# Autodesk Inventor assembly: SE. Chasis DC
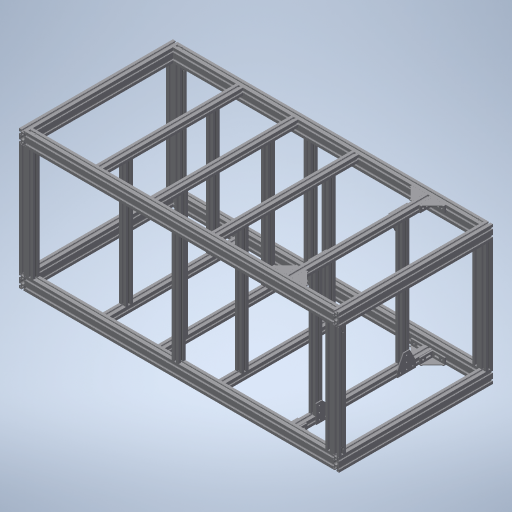
[picture p0: Inventor's stored thumbnail of the model, 512x512]
Saved by Autodesk Inventor 2024.2 (Build 282272000, 272)
## iProperties
Created: 2024-06-24
Part Number: SE. Chasis DC
Material: Genérico
Document SubType Name: Assembly
Designer: jd.castellanosq
Author: jd.castellanosq
## Documents named in this file (12)
- I:\MICROMECANICA\ALTAS ENERGIAS\Deteccion de Muones\Detectores centelladores\Partes Detector Centellador\SE Chasis DC\SE. Chasis DC.iam
- I:\MICROMECANICA\ALTAS ENERGIAS\Deteccion de Muones\Detectores centelladores\Partes Detectores centelladores\Chasis DC\Partes Chasis DC\Perfil 45X90.ipt
- I:\MICROMECANICA\ALTAS ENERGIAS\Deteccion de Muones\Detectores centelladores\Partes Detector Centellador\SE Chasis DC\Partes Chasis DC\Perfil 45X45\Perfil 45X45x910.ipt
- I:\MICROMECANICA\ALTAS ENERGIAS\Deteccion de Muones\Detectores centelladores\Partes Detectores centelladores\Chasis DC\Partes Chasis DC\Perfil 45X45.ipt
- I:\MICROMECANICA\ALTAS ENERGIAS\Deteccion de Muones\Detectores centelladores\Partes Detector Centellador\SE Chasis DC\Partes Chasis DC\Perfil 45X45\Perfil 45X45X720.ipt
- I:\MICROMECANICA\ALTAS ENERGIAS\Deteccion de Muones\Detectores centelladores\Partes Detector Centellador\SE Chasis DC\Partes Chasis DC\Accesorios perfileria\escuadra grande.ipt
- I:\MICROMECANICA\ALTAS ENERGIAS\Deteccion de Muones\Detectores centelladores\Partes Detector Centellador\SE Chasis DC\Partes Chasis DC\Accesorios perfileria\escuadra plana.ipt
- I:\MICROMECANICA\ALTAS ENERGIAS\Deteccion de Muones\Detectores centelladores\Partes Detector Centellador\SE Chasis DC\Partes Chasis DC\Accesorios perfileria\T.ipt
- I:\MICROMECANICA\ALTAS ENERGIAS\Deteccion de Muones\Detectores centelladores\Partes Detector Centellador\SE Chasis DC\Partes Chasis DC\Perfil 45X45\Perfil 45X45X810.ipt
- I:\MICROMECANICA\ALTAS ENERGIAS\Deteccion de Muones\Detectores centelladores\Partes Detector Centellador\SE Chasis DC\Partes Chasis DC\Perfil 45X90\Perfil 45X90x1000.ipt
- I:\MICROMECANICA\ALTAS ENERGIAS\Deteccion de Muones\Detectores centelladores\Partes Detector Centellador\SE Chasis DC\Partes Chasis DC\Perfil 45X90\Perfil 45X90x720.ipt
- I:\MICROMECANICA\ALTAS ENERGIAS\Deteccion de Muones\Detectores centelladores\Partes Detector Centellador\SE Chasis DC\Partes Chasis DC\Perfil 45X90\Perfil 45X90x1990.ipt
## Components (42 placed, 9 different names)
1. Perfil 45X90x1990:13 — Mate:65, Flush:83, Flush:84, Flush:85, Flush:86, Mate:66, Flush:92, Mate:71, Flush:94, Mate:72, Flush:108, Mate:82, Mate:91, Mate:99, Mate:114, Flush:131, Flush:138
2. Perfil 45X90x1000:17 — Mate:65, Flush:83, Flush:84, Flush:95, Flush:99, Mate:74
3. Perfil 45X90x1000:18 — Flush:85, Flush:86, Mate:66, Mate:67, Flush:87, Flush:88, Flush:93, Flush:97
4. Perfil 45X90x1990:21 — Mate:67, Flush:87, Flush:88, Flush:96, Mate:73, Flush:98, Flush:109, Flush:110, Mate:85, Mate:95, Mate:97, Mate:113, Flush:130, Mate:117
5. Perfil 45X45x910:39 — Flush:109
6. Perfil 45X45x910:40 — Flush:110, Mate:82
7. Perfil 45X45x910:41 — Flush:108, Flush:116, Mate:92, Mate:93, Mate:94, Flush:117, Mate:96, Flush:118, Mate:98, Flush:123, Flush:125
8. Perfil 45X45X810:45 — Flush:139
9. Perfil 45X45X810:46 — Flush:140
10. Perfil 45X45X810:47 — Mate:86, Mate:109, Mate:110, Mate:111
11. Perfil 45X45X810:48 — Mate:85, Mate:86, Mate:108, Flush:124, Mate:112, Flush:129
12. Perfil 45X45X810:49
13. Perfil 45X45X810:50
14. Perfil 45X90x1990:14 — Flush:106, Flush:107, Mate:78, Mate:101, Mate:102
15. Perfil 45X90x1000:19 — Flush:100, Flush:101, Mate:75, Mate:76, Flush:107, Mate:78
16. Perfil 45X90x1000:20 — Flush:103, Flush:104, Flush:105
17. Perfil 45X90x1990:28 — Mate:76, Flush:102, Mate:77, Flush:105, Flush:112, Mate:89, Mate:90, Mate:105, Mate:107, Mate:116
18. Perfil 45X90x720:9 — Flush:96, Flush:97, Mate:73, Flush:103, Flush:104
19. Perfil 45X90x720:10 — Flush:92, Mate:71, Flush:93
20. Perfil 45X90x720:11 — Flush:94, Mate:72, Flush:95, Flush:106
21. Perfil 45X90x720:12 — Flush:98, Flush:99, Mate:74, Flush:100, Flush:101, Mate:75, Flush:102, Mate:77
22. Perfil 45X45x910:42 — Mate:89
23. Perfil 45X45x910:43 — Flush:112, Flush:137
24. Perfil 45X45x910:44 — Mate:90, Flush:119, Mate:100, Flush:120, Mate:103, Flush:121, Mate:104, Flush:122, Mate:106, Flush:126, Flush:128
25. escuadra grande:1 — Flush:117, Mate:96, Mate:97
26. escuadra grande:2 — Mate:93, Mate:94, Mate:95
27. escuadra grande:3 — Flush:122, Mate:106, Mate:107
28. escuadra grande:4 — Flush:118, Mate:98, Mate:99
29. escuadra grande:5 — Flush:119, Mate:100, Mate:101
30. escuadra grande:6 — Flush:120, Mate:102, Mate:103
31. escuadra grande:7 — Flush:116, Mate:91, Mate:92
32. escuadra grande:8 — Flush:121, Mate:104, Mate:105
33. escuadra plana:1 — Mate:108, Flush:123, Flush:124
34. T:1 — Mate:111, Flush:126, Flush:127
35. T:2 — Mate:109, Flush:125, Mate:110, Flush:127
36. escuadra plana:2 — Mate:112, Flush:128, Flush:129
37. Perfil 45X45X720:51 — Mate:113, Flush:130
38. Perfil 45X45X720:52 — Mate:114, Flush:131
39. Perfil 45X45x910:53 — Flush:138, Mate:117
40. Perfil 45X45x910:54 — Flush:137, Mate:116
41. Perfil 45X45X810:55 — Flush:139
42. Perfil 45X45X810:56 — Flush:140
## Relationships (122: Flush 68, Mate 54)
- [Mate]: Perfil 45X90x1990:13
- [Mate]: Perfil 45X90x1990:13
- [Flush]: Perfil 45X90x1990:13
- [Flush]: Perfil 45X45X810:47 ↔ Perfil 45X45X810:48
- [Flush]: Perfil 45X45X810:47 ↔ Perfil 45X45X810:48
- [Flush]: Perfil 45X45X810:45 ↔ Perfil 45X45X810:46
- [Flush]: Perfil 45X45X810:45 ↔ Perfil 45X45X810:46
- [Flush]: Perfil 45X45x910:41 ↔ Perfil 45X45X810:48
- [Flush]: Perfil 45X45X810:45 ↔ Perfil 45X45X810:48
- [Flush]: Perfil 45X45X810:46 ↔ Perfil 45X45X810:47
- [Flush]: Perfil 45X45x910:39 ↔ Perfil 45X45X810:50
- [Flush]: Perfil 45X45X810:48 ↔ Perfil 45X45X810:50
- [Flush]: Perfil 45X45x910:39 ↔ Perfil 45X45X810:49
- [Flush]: Perfil 45X45X810:47 ↔ Perfil 45X45X810:49
- [Mate]: Perfil 45X45X810:50 ↔ Perfil 45X45x910:42
- [Flush]: Perfil 45X45X810:50 ↔ Perfil 45X45x910:42
- [Mate]: Perfil 45X90x1990:28 ↔ Perfil 45X45x910:43
- [Flush]: Perfil 45X45X810:45 ↔ Perfil 45X45x910:43
- [Mate]: Perfil 45X45X810:48 ↔ Perfil 45X45x910:44
- [Flush]: Perfil 45X45X810:48 ↔ Perfil 45X45x910:44
- Mate:65: Perfil 45X90x1990:13 ↔ Perfil 45X90x1000:17
- Flush:83: Perfil 45X90x1990:13 ↔ Perfil 45X90x1000:17
- Flush:84: Perfil 45X90x1990:13 ↔ Perfil 45X90x1000:17
- Flush:85: Perfil 45X90x1990:13 ↔ Perfil 45X90x1000:18
- Flush:86: Perfil 45X90x1990:13 ↔ Perfil 45X90x1000:18
- Mate:66: Perfil 45X90x1990:13 ↔ Perfil 45X90x1000:18
- Mate:67: Perfil 45X90x1000:18 ↔ Perfil 45X90x1990:21
- Flush:87: Perfil 45X90x1000:18 ↔ Perfil 45X90x1990:21
- Flush:88: Perfil 45X90x1000:18 ↔ Perfil 45X90x1990:21
- [Mate]: Perfil 45X90x1990:13 ↔ Perfil 45X45x910:39
- [Mate]: Perfil 45X90x1990:13 ↔ Perfil 45X45x910:41
- Flush:92: Perfil 45X90x1990:13 ↔ Perfil 45X90x720:10
- Mate:71: Perfil 45X90x1990:13 ↔ Perfil 45X90x720:10
- Flush:93: Perfil 45X90x1000:18 ↔ Perfil 45X90x720:10
- Flush:94: Perfil 45X90x1990:13 ↔ Perfil 45X90x720:11
- Mate:72: Perfil 45X90x1990:13 ↔ Perfil 45X90x720:11
- Flush:95: Perfil 45X90x1000:17 ↔ Perfil 45X90x720:11
- Flush:96: Perfil 45X90x1990:21 ↔ Perfil 45X90x720:9
- Flush:97: Perfil 45X90x1000:18 ↔ Perfil 45X90x720:9
- Mate:73: Perfil 45X90x1990:21 ↔ Perfil 45X90x720:9
- Flush:98: Perfil 45X90x1990:21 ↔ Perfil 45X90x720:12
- Flush:99: Perfil 45X90x1000:17 ↔ Perfil 45X90x720:12
- Mate:74: Perfil 45X90x1000:17 ↔ Perfil 45X90x720:12
- Flush:100: Perfil 45X90x1000:19 ↔ Perfil 45X90x720:12
- Flush:101: Perfil 45X90x1000:19 ↔ Perfil 45X90x720:12
- Mate:75: Perfil 45X90x1000:19 ↔ Perfil 45X90x720:12
- Mate:76: Perfil 45X90x1000:19 ↔ Perfil 45X90x1990:28
- Flush:102: Perfil 45X90x1990:28 ↔ Perfil 45X90x720:12
- Mate:77: Perfil 45X90x1990:28 ↔ Perfil 45X90x720:12
- Flush:103: Perfil 45X90x1000:20 ↔ Perfil 45X90x720:9
- Flush:104: Perfil 45X90x1000:20 ↔ Perfil 45X90x720:9
- Flush:105: Perfil 45X90x1000:20 ↔ Perfil 45X90x1990:28
- Flush:106: Perfil 45X90x1990:14 ↔ Perfil 45X90x720:11
- Flush:107: Perfil 45X90x1990:14 ↔ Perfil 45X90x1000:19
- Mate:78: Perfil 45X90x1990:14 ↔ Perfil 45X90x1000:19
- Flush:108: Perfil 45X90x1990:13 ↔ Perfil 45X45x910:41
- [Mate]: Perfil 45X45x910:41 ↔ Perfil 45X45X810:47
- Flush:109: Perfil 45X90x1990:21 ↔ Perfil 45X45x910:39
- [Mate]: Perfil 45X45x910:39 ↔ Perfil 45X45X810:50
- [Mate]: Perfil 45X45x910:39 ↔ Perfil 45X45X810:49
- Flush:110: Perfil 45X90x1990:21 ↔ Perfil 45X45x910:40
- Mate:82: Perfil 45X90x1990:13 ↔ Perfil 45X45x910:40
- [Mate]: Perfil 45X45x910:40 ↔ Perfil 45X45X810:46
- [Flush]: Perfil 45X45x910:40 ↔ Perfil 45X45X810:46
- Flush:112: Perfil 45X90x1990:28 ↔ Perfil 45X45x910:43
- [Flush]: Perfil 45X45X810:45 ↔ Perfil 45X45x910:43
- Mate:85 (150 mm): Perfil 45X90x1990:21 ↔ Perfil 45X45X810:48
- Mate:86 (-610 mm): Perfil 45X45X810:47 ↔ Perfil 45X45X810:48
- Mate:89: Perfil 45X90x1990:28 ↔ Perfil 45X45x910:42
- Mate:90: Perfil 45X90x1990:28 ↔ Perfil 45X45x910:44
- Flush:116: Perfil 45X45x910:41 ↔ escuadra grande:7
- Mate:91: Perfil 45X90x1990:13 ↔ escuadra grande:7
- Mate:92: Perfil 45X45x910:41 ↔ escuadra grande:7
- Mate:93: Perfil 45X45x910:41 ↔ escuadra grande:2
- Mate:94: Perfil 45X45x910:41 ↔ escuadra grande:2
- Mate:95: Perfil 45X90x1990:21 ↔ escuadra grande:2
- Flush:117: Perfil 45X45x910:41 ↔ escuadra grande:1
- Mate:96: Perfil 45X45x910:41 ↔ escuadra grande:1
- Mate:97: Perfil 45X90x1990:21 ↔ escuadra grande:1
- Flush:118: Perfil 45X45x910:41 ↔ escuadra grande:4
- Mate:98: Perfil 45X45x910:41 ↔ escuadra grande:4
- Mate:99: Perfil 45X90x1990:13 ↔ escuadra grande:4
- Flush:119: Perfil 45X45x910:44 ↔ escuadra grande:5
- Mate:100: Perfil 45X45x910:44 ↔ escuadra grande:5
- Mate:101: Perfil 45X90x1990:14 ↔ escuadra grande:5
- Flush:120: Perfil 45X45x910:44 ↔ escuadra grande:6
- Mate:102: Perfil 45X90x1990:14 ↔ escuadra grande:6
- Mate:103: Perfil 45X45x910:44 ↔ escuadra grande:6
- Flush:121: Perfil 45X45x910:44 ↔ escuadra grande:8
- Mate:104: Perfil 45X45x910:44 ↔ escuadra grande:8
- Mate:105: Perfil 45X90x1990:28 ↔ escuadra grande:8
- Flush:122: Perfil 45X45x910:44 ↔ escuadra grande:3
- Mate:106: Perfil 45X45x910:44 ↔ escuadra grande:3
- Mate:107: Perfil 45X90x1990:28 ↔ escuadra grande:3
- Mate:108: Perfil 45X45X810:48 ↔ escuadra plana:1
- Flush:123: Perfil 45X45x910:41 ↔ escuadra plana:1
- Flush:124: Perfil 45X45X810:48 ↔ escuadra plana:1
- Mate:109: Perfil 45X45X810:47 ↔ T:2
- Flush:125: Perfil 45X45x910:41 ↔ T:2
- Mate:110 (-2.5 mm): Perfil 45X45X810:47 ↔ T:2
- Mate:111: Perfil 45X45X810:47 ↔ T:1
- Flush:126: Perfil 45X45x910:44 ↔ T:1
- Flush:127: T:1 ↔ T:2
- Mate:112: Perfil 45X45X810:48 ↔ escuadra plana:2
- Flush:128: Perfil 45X45x910:44 ↔ escuadra plana:2
- Flush:129: Perfil 45X45X810:48 ↔ escuadra plana:2
- Mate:113: Perfil 45X90x1990:21 ↔ Perfil 45X45X720:51
- Flush:130: Perfil 45X90x1990:21 ↔ Perfil 45X45X720:51
- Mate:114: Perfil 45X90x1990:13 ↔ Perfil 45X45X720:52
- Flush:131: Perfil 45X90x1990:13 ↔ Perfil 45X45X720:52
- [Flush]: Perfil 45X45X810:55 ↔ Perfil 45X45X810:56
- [Flush]: Perfil 45X45X810:55 ↔ Perfil 45X45X810:56
- [Flush]: Perfil 45X45x910:54 ↔ Perfil 45X45X810:55
- [Mate]: Perfil 45X45x910:53 ↔ Perfil 45X45X810:56
- [Flush]: Perfil 45X45x910:53 ↔ Perfil 45X45X810:56
- [Flush]: Perfil 45X45x910:54 ↔ Perfil 45X45X810:55
- Flush:137: Perfil 45X45x910:43 ↔ Perfil 45X45x910:54
- Mate:116: Perfil 45X90x1990:28 ↔ Perfil 45X45x910:54
- Flush:138: Perfil 45X90x1990:13 ↔ Perfil 45X45x910:53
- Mate:117: Perfil 45X90x1990:21 ↔ Perfil 45X45x910:53
- Flush:139: Perfil 45X45X810:45 ↔ Perfil 45X45X810:55
- Flush:140: Perfil 45X45X810:46 ↔ Perfil 45X45X810:56
## Named parameters: d361_d307 = 0 mm, d362_d304 = 0 mm, d363_d305 = 0 mm, d364_d222 = 0 mm, d365_d177 = 0 mm, d366_d178 = 0 mm
